# Autodesk Inventor assembly: Assembly HC-05
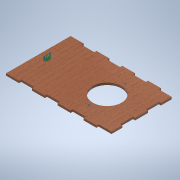
[picture p0: Inventor's stored thumbnail of the model, 180x180]
Saved by Autodesk Inventor 2021 (Build 250183000, 183)
## iProperties
Manager: Pierloot J.
Company: Emmaüs Bovenbouw Aalter
Created: 2021-01-30
Part Number: Assembly HC-05
Catalog Web Link: http://emmausbovenbouw.op-weg.be/
Vendor: Emmaüs Bovenbouw Aalter
Document SubType Name: Assembly
Designer: Antho
Engineer: Declercq St.
Authority: Declercq St.
Title: Algemene Projecttitel
Author: Antho
## Documents named in this file (3)
- F:\GIP 6EM\Assembly\Assembly HC-05.iam
- F:\GIP 6EM\Frame\Plaat boven.ipt
- F:\GIP 6EM\Bevestigingen\HC-05.ipt
## Components (2 placed, 2 different names)
1. Plaat boven:1 — Mate:1, Flush:1, Mate:2
2. HC-05:1 — Mate:1, Flush:1, Mate:2
## Relationships (3: Mate 2, Flush 1)
- Mate:1: Plaat boven:1 ↔ HC-05:1
- Flush:1 (-10 mm): Plaat boven:1 ↔ HC-05:1
- Mate:2: Plaat boven:1 ↔ HC-05:1
